# Autodesk Inventor assembly: kolo
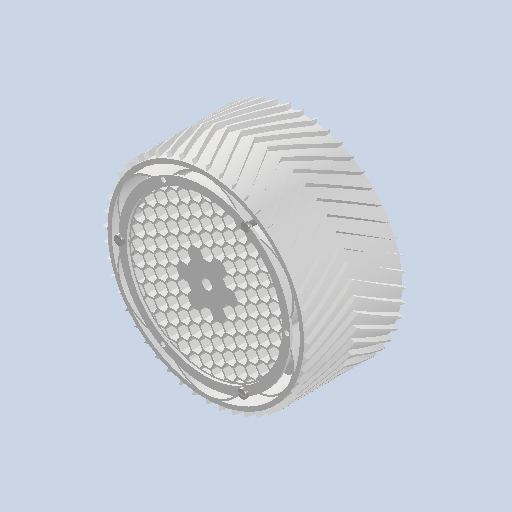
[picture p0: Inventor's stored thumbnail of the model, 512x512]
Saved by Autodesk Inventor 2025.3 (Build 293356000, 356)
## iProperties
Created: 2026-04-01
Part Number: kolo
Document SubType Name: Assembly
Designer: ksawe
Author: ksawe
## Documents named in this file (5)
- C:\Users\ksawe\OneDrive\Pulpit\Exomy v1\wersja2\kolo.iam
- C:\Users\ksawe\OneDrive\Pulpit\Exomy v1\wersja2\felga.ipt
- C:\Users\ksawe\Downloads\opona_nowa\opona_nowa\opona_nowa.ipt
- C:\Users\ksawe\OneDrive\Pulpit\Exomy v1\wersja2\bead lock.ipt
- C:\Users\ksawe\OneDrive\Dokumenty\Inventor\Content Center Files\R2025\en-US\PN-85 M-82219\PN-85_M-82219 - M3 x 25 - 0,5.ipt
## Components (10 placed, 4 different names)
1. opona_nowa:1 — Mate:1
2. felga:1 — Mate:1, Tangent:1, Tangent:2, Mate:2, Tangent:3, Tangent:4, Mate:3
3. bead lock:1 — Tangent:1, Tangent:2, Mate:2, Insert:4, Insert:5, Insert:6
4. bead lock:2 — Tangent:3, Tangent:4, Mate:3, Insert:1, Insert:2, Insert:3
5. PN-85/M-82219 M3 x 25:1 — Insert:1
6. PN-85/M-82219 M3 x 25:2 — Insert:3
7. PN-85/M-82219 M3 x 25:3 — Insert:5
8. PN-85/M-82219 M3 x 25:4 — Insert:2
9. PN-85/M-82219 M3 x 25:5 — Insert:6
10. PN-85/M-82219 M3 x 25:6 — Insert:4
## Relationships (13: Insert 6, Tangent 4, Mate 3)
- Mate:1: opona_nowa:1 ↔ felga:1
- Tangent:1: felga:1 ↔ bead lock:1
- Tangent:2: felga:1 ↔ bead lock:1
- Mate:2: felga:1 ↔ bead lock:1
- Tangent:3: felga:1 ↔ bead lock:2
- Tangent:4: felga:1 ↔ bead lock:2
- Mate:3: felga:1 ↔ bead lock:2
- Insert:1: bead lock:2 ↔ PN-85/M-82219 M3 x 25:1
- Insert:2: bead lock:2 ↔ PN-85/M-82219 M3 x 25:4
- Insert:3: bead lock:2 ↔ PN-85/M-82219 M3 x 25:2
- Insert:4: bead lock:1 ↔ PN-85/M-82219 M3 x 25:6
- Insert:5: bead lock:1 ↔ PN-85/M-82219 M3 x 25:3
- Insert:6: bead lock:1 ↔ PN-85/M-82219 M3 x 25:5
